# Autodesk Inventor assembly: holder 2.611
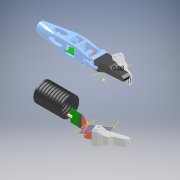
[picture p0: Inventor's stored thumbnail of the model, 180x180]
Saved by Autodesk Inventor 2019 (Build 230136000, 136)
## iProperties
Created: 2020-03-27
Part Number: holder 2.611
Document SubType Name: Assembly
Designer: Thomas Zhihao Luo
Author: Thomas Zhihao Luo
## Documents named in this file (10)
- C:\Users\Thomas Zhihao Luo\Documents\chronic_neuropixels\2.611\holder 2.611.iam
- C:\Users\Thomas Zhihao Luo\Documents\chronic_neuropixels\2.611\premade_implant.iam
- C:\Users\Thomas Zhihao Luo\Documents\chronic_neuropixels\2.611\headstage+flex connector.iam
- C:\Users\Thomas Zhihao Luo\Documents\chronic_neuropixels\2.611\flexcable6.ipt
- C:\Users\Thomas Zhihao Luo\Documents\chronic_neuropixels\2.611\assembled_implant.ipt
- C:\Users\Thomas Zhihao Luo\Documents\chronic_neuropixels\2.611\Part82.ipt
- C:\Users\Thomas Zhihao Luo\Documents\chronic_neuropixels\2.611\headstage+flex connector_MIR.iam
- C:\Users\Thomas Zhihao Luo\Documents\chronic_neuropixels\2.611\assembled_implant_MIR.ipt
- C:\Users\Thomas Zhihao Luo\Documents\chronic_neuropixels\2.611\Part82_MIR.ipt
- C:\Users\Thomas Zhihao Luo\Documents\chronic_neuropixels\2.611\Part6.ipt
## Components (10 placed, 9 different names)
1. premade_implant:1 [sub-assembly] — Mate:7
2. headstage+flex connector:1 [sub-assembly] — Flush:6, Flush:9, Flush:10
3. headstage+flex connector:2 [sub-assembly]
4. flexcable6:1 — Flush:2, Flush:3, Flush:4
5. assembled_implant:3 — Angle:1, Angle:2, Mate:3, Angle:4, Flush:7, Flush:8, Flush:11
6. flex cable — Flush:6, Flush:7, Flush:8, Flush:9, Flush:10, Flush:11
7. headstage+flex connector_MIR:1 [sub-assembly] — Mate:16, Mate:17, Mate:20
8. assembled_implant_MIR:1 — Angle:5, Angle:6, Mate:13, Angle:7, Mate:15, Mate:18, Mate:19
9. flex cable MIR — Mate:15, Mate:16, Mate:17, Mate:18, Mate:19, Mate:20
10. Part6:1
## Relationships (30: Mate 14, Flush 9, Angle 7)
- Flush:2: flexcable6:1
- Flush:3: flexcable6:1
- Flush:4: flexcable6:1
- Angle:1 (0 deg): assembled_implant:3
- Angle:2 (20 deg): assembled_implant:3
- Angle:3 (0 deg)
- Mate:3: assembled_implant:3
- Mate:4
- Mate:7: premade_implant:1
- Mate:10
- Mate:11
- Angle:4 (0 deg): assembled_implant:3
- Mate:12 (4 mm)
- Flush:6: headstage+flex connector:1 ↔ flex cable
- Flush:7: assembled_implant:3 ↔ flex cable
- Flush:8: assembled_implant:3 ↔ flex cable
- Flush:9: headstage+flex connector:1 ↔ flex cable
- Flush:10: headstage+flex connector:1 ↔ flex cable
- Flush:11: assembled_implant:3 ↔ flex cable
- Angle:5 (-20 deg): assembled_implant_MIR:1
- Angle:6 (0 deg): assembled_implant_MIR:1
- Mate:13: assembled_implant_MIR:1
- Angle:7 (0 deg): assembled_implant_MIR:1
- Mate:14
- Mate:15: assembled_implant_MIR:1 ↔ flex cable MIR
- Mate:16: headstage+flex connector_MIR:1 ↔ flex cable MIR
- Mate:17: headstage+flex connector_MIR:1 ↔ flex cable MIR
- Mate:18: assembled_implant_MIR:1 ↔ flex cable MIR
- Mate:19: assembled_implant_MIR:1 ↔ flex cable MIR
- Mate:20: headstage+flex connector_MIR:1 ↔ flex cable MIR
